# Autodesk Inventor assembly: Assembly completo
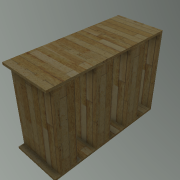
[picture p0: Inventor's stored thumbnail of the model, 180x180]
Saved by Autodesk Inventor 2015 (Build 190159000, 159)
## iProperties
Created: 2016-01-26
Part Number: Assembly completo
Document SubType Name: Assembly
Designer: iberopuebla
Author: iberopuebla
## Documents named in this file (3)
- H:\3d\Assembly completo.iam
- H:\3d\Assembly cajon.iam
- H:\3d\Assembly mueble.iam
## Components (4 placed, 2 different names)
1. Assembly cajon:1 [sub-assembly] — Mate:2, Mate:4, Flush:2, Mate:6
2. Assembly cajon:2 [sub-assembly] — Mate:1, Flush:3, Mate:5
3. Assembly mueble:2 [sub-assembly] — Mate:1, Mate:2, Mate:3, Mate:4, Flush:1, Flush:2, Flush:3, Mate:5, Mate:6, Mate:7
4. Assembly cajon:3 [sub-assembly] — Mate:3, Flush:1, Mate:7
## Relationships (10: Mate 7, Flush 3)
- Mate:1: Assembly cajon:2 ↔ Assembly mueble:2
- Mate:2: Assembly cajon:1 ↔ Assembly mueble:2
- Mate:3: Assembly mueble:2 ↔ Assembly cajon:3
- Mate:4: Assembly cajon:1 ↔ Assembly mueble:2
- Flush:1: Assembly mueble:2 ↔ Assembly cajon:3
- Flush:2: Assembly cajon:1 ↔ Assembly mueble:2
- Flush:3: Assembly cajon:2 ↔ Assembly mueble:2
- Mate:5 (2 mm): Assembly cajon:2 ↔ Assembly mueble:2
- Mate:6 (2 mm): Assembly cajon:1 ↔ Assembly mueble:2
- Mate:7 (2 mm): Assembly mueble:2 ↔ Assembly cajon:3
